# Autodesk Inventor assembly: derive_rod_v7
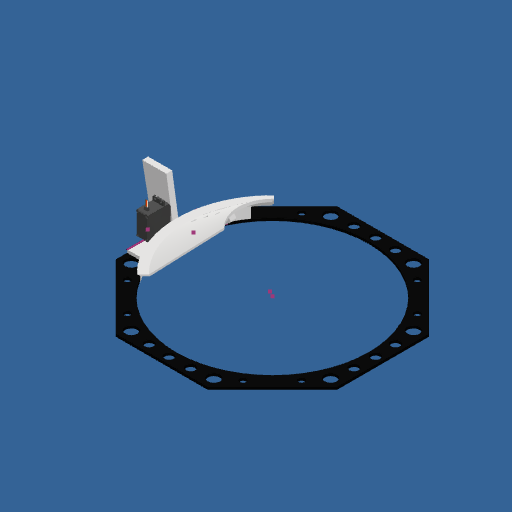
[picture p0: Inventor's stored thumbnail of the model, 512x512]
Saved by Autodesk Inventor 2026.2 (Build 302298000, 298)
## iProperties
Created: 2026-01-13
Part Number: derive_rod_v7
Document SubType Name: Assembly
Designer: Thoma
Author: Thoma
## Documents named in this file (6)
- C:\Users\Thoma\OneDrive\Desktop\dir\telescope_cover\cover\derive_rod_v9.iam
- C:\Users\Thoma\OneDrive\Desktop\dir\telescope_cover\telescope\version_3\Telescope_End.ipt
- C:\Users\Thoma\OneDrive\Desktop\dir\telescope_cover\cover\Cover_Upper_v3.ipt
- C:\Users\Thoma\OneDrive\Desktop\dir\telescope_cover\cover\Base_Plate_v2.ipt
- C:\Users\Thoma\OneDrive\Desktop\dir\telescope_cover\servo\DSS-M15S Servo.ipt
- C:\Users\Thoma\OneDrive\Desktop\dir\telescope_cover\cover\rod_v7.1.ipt
## Components (5 placed, 5 different names)
1. Telescope_End:1 — Mate:1, Mate:2, Angle:4, Mate:3, Mate:4, Mate:5, Flush:1
2. Cover_Upper_v3:1 — Mate:1, Mate:2, Angle:4, Mate:7, Mate:8, Tangent:1
3. Base_Plate_v2:1 — Mate:3, Mate:4, Mate:5, Mate:6, Flush:8
4. DSS-M15S Servo:1 — Mate:6, Flush:1, Flush:8
5. rod_v7.1:1 — Mate:7, Mate:8, Tangent:1
## Relationships (12: Mate 8, Flush 2, Angle 1, Tangent 1)
- Mate:1: Telescope_End:1 ↔ Cover_Upper_v3:1
- Mate:2 (1.977 mm): Telescope_End:1 ↔ Cover_Upper_v3:1
- Angle:4 (45 deg): Telescope_End:1 ↔ Cover_Upper_v3:1
- Mate:3: Telescope_End:1 ↔ Base_Plate_v2:1
- Mate:4: Telescope_End:1 ↔ Base_Plate_v2:1
- Mate:5: Telescope_End:1 ↔ Base_Plate_v2:1
- Mate:6 (14 mm): Base_Plate_v2:1 ↔ DSS-M15S Servo:1
- Flush:1 (2.5 mm): Telescope_End:1 ↔ DSS-M15S Servo:1
- Flush:8 (13.475 mm): Base_Plate_v2:1 ↔ DSS-M15S Servo:1
- Mate:7: Cover_Upper_v3:1 ↔ rod_v7.1:1
- Mate:8: Cover_Upper_v3:1 ↔ rod_v7.1:1
- Tangent:1 (-1 mm): Cover_Upper_v3:1 ↔ rod_v7.1:1
